# Autodesk Inventor assembly: completeassembly
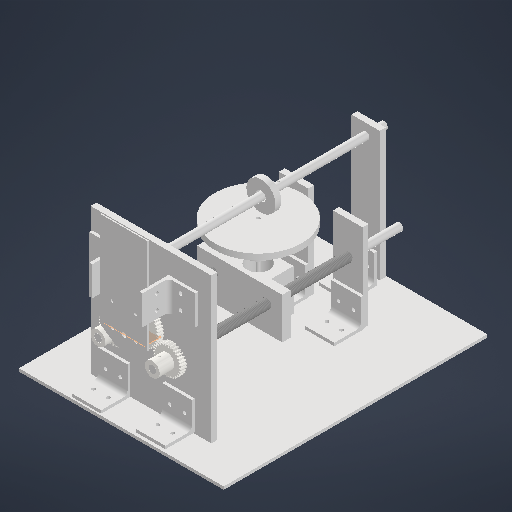
[picture p0: Inventor's stored thumbnail of the model, 512x512]
Saved by Autodesk Inventor 2026.1 (Build 301233000, 233)
## iProperties
Created: 2025-11-11
Part Number: completeassembly
Document SubType Name: Assembly
Designer: Mukund Advaith
Author: Mukund Advaith
## Documents named in this file (17)
- C:\Users\mukun\Downloads\project\finalreport\completeassembly.iam
- C:\Users\mukun\Downloads\project\finalreport\base.ipt
- C:\Users\mukun\Downloads\project\finalreport\bigwall.ipt
- C:\Users\mukun\Downloads\project\finalreport\spur1.iam
- C:\Users\mukun\Downloads\project\finalreport\spur2.iam
- C:\Users\mukun\Downloads\project\finalreport\driveshaft1.ipt
- C:\Users\mukun\Downloads\project\finalreport\driveshaft2.ipt
- C:\Users\mukun\Downloads\project\finalreport\carriage.ipt
- C:\Users\mukun\Downloads\project\finalreport\tallwall1.ipt
- C:\Users\mukun\Downloads\project\finalreport\tallwall3.ipt
- C:\Users\mukun\Downloads\project\finalreport\stationaryrod.ipt
- C:\Users\mukun\Downloads\project\finalreport\tallwall2.ipt
- C:\Users\mukun\Downloads\project\finalreport\lclamp.ipt
- C:\Users\mukun\Downloads\project\finalreport\Project_Rough_disc.ipt
- C:\Users\mukun\Downloads\project\finalreport\Project_Stationary_Wheel.ipt
- C:\Users\mukun\Downloads\project\finalreport\waste.ipt
- C:\Users\mukun\Downloads\project\finalreport\motorholder.ipt
## Components (23 placed, 16 different names)
1. base:1 — Mate:11
2. bigwall:1 — Mate:1, Mate:2, Mate:3, Mate:4, Mate:5, Mate:6, Mate:11, Mate:14, Mate:15, Mate:17, Mate:18, Mate:27, Mate:28
3. spur1:1 [sub-assembly] — Mate:1, Mate:2, Mate:9
4. spur1:2 [sub-assembly] — Mate:3, Mate:4, Mate:7, Mate:8
5. spur2:1 [sub-assembly] — Mate:5, Mate:6, Mate:25, Mate:26
6. driveshaft1:1 — Mate:7, Mate:8, Mate:10, Mate:12
7. driveshaft2:1 — Mate:9, Mate:13
8. carriage:1 — Mate:10, Mate:22
9. tallwall1:1 — Mate:12, Mate:19
10. tallwall3:1 — Mate:13, Mate:20
11. stationaryrod:1 — Mate:14, Mate:15, Mate:16, Mate:23
12. tallwall2:1 — Mate:16, Mate:21
13. lclamp:1 — Mate:17
14. lclamp:2 — Mate:18
15. lclamp:3 — Mate:19
16. lclamp:4 — Mate:20
17. lclamp:5 — Mate:21
18. Project_Rough_disc:1 — Mate:22, Mate:24
19. Project_Stationary_Wheel:1 — Mate:23
20. waste:1 — Mate:24
21. motorholder:1 — Mate:25, Mate:26
22. lclamp:6 — Mate:27
23. lclamp:7 — Mate:28
## Relationships (28: Mate 28)
- Mate:1: bigwall:1 ↔ spur1:1
- Mate:2: bigwall:1 ↔ spur1:1
- Mate:3: bigwall:1 ↔ spur1:2
- Mate:4: bigwall:1 ↔ spur1:2
- Mate:5: bigwall:1 ↔ spur2:1
- Mate:6: bigwall:1 ↔ spur2:1
- Mate:7: spur1:2 ↔ driveshaft1:1
- Mate:8: spur1:2 ↔ driveshaft1:1
- Mate:9: spur1:1 ↔ driveshaft2:1
- Mate:10: driveshaft1:1 ↔ carriage:1
- Mate:11: base:1 ↔ bigwall:1
- Mate:12: driveshaft1:1 ↔ tallwall1:1
- Mate:13: driveshaft2:1 ↔ tallwall3:1
- Mate:14: bigwall:1 ↔ stationaryrod:1
- Mate:15: bigwall:1 ↔ stationaryrod:1
- Mate:16: stationaryrod:1 ↔ tallwall2:1
- Mate:17: bigwall:1 ↔ lclamp:1
- Mate:18: bigwall:1 ↔ lclamp:2
- Mate:19: tallwall1:1 ↔ lclamp:3
- Mate:20: tallwall3:1 ↔ lclamp:4
- Mate:21: tallwall2:1 ↔ lclamp:5
- Mate:22: carriage:1 ↔ Project_Rough_disc:1
- Mate:23: stationaryrod:1 ↔ Project_Stationary_Wheel:1
- Mate:24: Project_Rough_disc:1 ↔ waste:1
- Mate:25: spur2:1 ↔ motorholder:1
- Mate:26: spur2:1 ↔ motorholder:1
- Mate:27: bigwall:1 ↔ lclamp:6
- Mate:28: bigwall:1 ↔ lclamp:7
